# Autodesk Inventor assembly: Z Motor Unit B
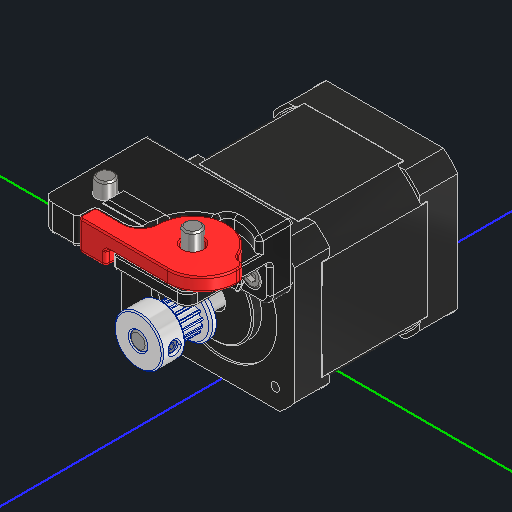
[picture p0: Inventor's stored thumbnail of the model, 512x512]
Saved by Autodesk Inventor 2022.2 (Build 262287010, 287A)
## iProperties
Created: 2022-03-12
Part Number: Z Motor Unit B
Document SubType Name: Assembly
Designer: sleib
Author: sleib
## Documents named in this file (7)
- C:\Users\sleib\Projekte\Voron-2\CAD\Inventor\Z Motor-Unit [B].iam
- C:\Users\sleib\Projekte\Voron-2\CAD\Inventor\NEMA17 Black.ipt
- C:\Users\sleib\Projekte\Voron-2\CAD\Inventor\GT2 16T Pulley (6mm).ipt
- C:\Users\sleib\Projekte\Voron-2\CAD\Inventor\Z Motor-Mount [B].ipt
- C:\Users\sleib\Projekte\Voron-2\CAD\Inventor\M3x8 SHCS.ipt
- C:\Users\sleib\Projekte\Voron-2\CAD\Inventor\Z Belt-Tensioner [B].ipt
- C:\Users\sleib\Projekte\Voron-2\CAD\Inventor\M5x10 BHCS.ipt
## Components (9 placed, 6 different names)
1. NEMA17 Black:1 — Passend:1, Fluchtend:1, Passend:2, Passend:5, Passend:6, Passend:7
2. GT2 16T Pulley (6mm):1 — Passend:1, Fluchtend:1
3. Z Motor Mount B:1 — Passend:2, Passend:18, Passend:19, Passend:20, Passend:8, Passend:9, Passend:10, Passend:12, Passend:13, Passend:14, Passend:15, Passend:16
4. Z Belt-Tensioner [B]:1 — Passend:12, Passend:17
5. M3x8 SHCS:1 — Passend:7, Passend:10, Passend:19
6. M3x8 SHCS:2 — Passend:6, Passend:18, Passend:8
7. M3x8 SHCS:3 — Passend:5, Passend:9, Passend:20
8. M5x10 BHCS:1 — Passend:13, Passend:15
9. M5x10 BHCS:2 — Passend:14, Passend:16, Passend:17
## Relationships (18: Mate 17, Flush 1)
- Passend:1 [Mate]: NEMA17 Black:1 ↔ GT2 16T Pulley (6mm):1
- Fluchtend:1 [Flush]: NEMA17 Black:1 ↔ GT2 16T Pulley (6mm):1
- Passend:2 [Mate]: NEMA17 Black:1 ↔ Z Motor Mount B:1
- Passend:5 [Mate]: NEMA17 Black:1 ↔ M3x8 SHCS:3
- Passend:6 [Mate]: NEMA17 Black:1 ↔ M3x8 SHCS:2
- Passend:7 [Mate]: NEMA17 Black:1 ↔ M3x8 SHCS:1
- Passend:18 [Mate]: Z Motor Mount B:1 ↔ M3x8 SHCS:2
- Passend:19 [Mate]: Z Motor Mount B:1 ↔ M3x8 SHCS:1
- Passend:20 [Mate]: Z Motor Mount B:1 ↔ M3x8 SHCS:3
- Passend:8 [Mate]: Z Motor Mount B:1 ↔ M3x8 SHCS:2
- Passend:9 [Mate]: Z Motor Mount B:1 ↔ M3x8 SHCS:3
- Passend:10 [Mate]: Z Motor Mount B:1 ↔ M3x8 SHCS:1
- Passend:12 [Mate]: Z Motor Mount B:1 ↔ Z Belt-Tensioner [B]:1
- Passend:13 [Mate]: Z Motor Mount B:1 ↔ M5x10 BHCS:1
- Passend:14 [Mate]: Z Motor Mount B:1 ↔ M5x10 BHCS:2
- Passend:15 [Mate]: Z Motor Mount B:1 ↔ M5x10 BHCS:1
- Passend:16 [Mate]: Z Motor Mount B:1 ↔ M5x10 BHCS:2
- Passend:17 [Mate]: Z Belt-Tensioner [B]:1 ↔ M5x10 BHCS:2
